# Autodesk Inventor assembly: pot1_assy
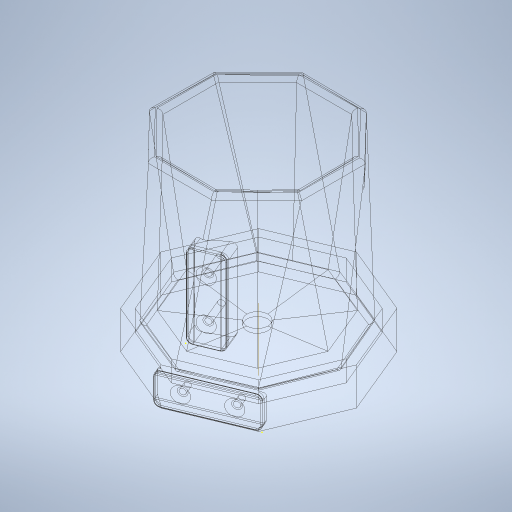
[picture p0: Inventor's stored thumbnail of the model, 512x512]
Saved by Autodesk Inventor 2023 (Build 270158000, 158)
## iProperties
Created: 2025-10-09
Part Number: pot1_assy
Document SubType Name: Assembly
Designer: Justin Pascual
Author: Justin Pascual
## Documents named in this file (4)
- C:\Users\Justin Pascual\Documents\GitHub\modular-flower-pot\pot1_assy.iam
- C:\Users\Justin Pascual\Documents\GitHub\modular-flower-pot\pot1.ipt
- C:\Users\Justin Pascual\Documents\GitHub\modular-flower-pot\dovetail.ipt
- C:\Users\Justin Pascual\Documents\GitHub\modular-flower-pot\base1.ipt
## Components (4 placed, 3 different names)
1. pot1:1 — Mate:7, Mate:8, Flush:10, Flush:11, Mate:10, Mate:11
2. dovetail:1 — Mate:7, Mate:8, Mate:11
3. base1:1 — Flush:10, Flush:11, Mate:10, Mate:12, Mate:13, Mate:14
4. dovetail:2 — Mate:12, Mate:13, Mate:14
## Relationships (9: Mate 7, Flush 2)
- Mate:7: pot1:1 ↔ dovetail:1
- Mate:8: pot1:1 ↔ dovetail:1
- Flush:10: pot1:1 ↔ base1:1
- Flush:11 (16.51 mm): pot1:1 ↔ base1:1
- Mate:10 (16.51 mm): pot1:1 ↔ base1:1
- Mate:11: pot1:1 ↔ dovetail:1
- Mate:12: base1:1 ↔ dovetail:2
- Mate:13: base1:1 ↔ dovetail:2
- Mate:14: base1:1 ↔ dovetail:2
